# Autodesk Inventor assembly: head_v2
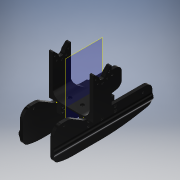
[picture p0: Inventor's stored thumbnail of the model, 180x180]
Saved by Autodesk Inventor 2018 (Build 220112000, 112)
## iProperties
Created: 2020-02-17
Part Number: head_v2
Document SubType Name: Assembly
Designer: bitbots
Author: bitbots
## Documents named in this file (4)
- C:\Users\bitbots\Desktop\bitbots_hardware\wolfgang\assembly\head\head_v2.iam
- C:\Users\bitbots\Desktop\bitbots_hardware\wolfgang\assembly\head\camera_lower_baseler_wolfgang_v2.1.ipt
- C:\Users\bitbots\Desktop\bitbots_hardware\wolfgang\assembly\head\camera_side_basler_wolfgang_v2.2.ipt
- C:\Users\bitbots\Desktop\bitbots_hardware\wolfgang\assembly\head\camera_side_basler_wolfgang_v2.2_MIR1.ipt
## Components (3 placed, 3 different names)
1. camera_lower_baseler_wolfgang_v2.1:1 — Mate:1, Mate:2, Mate:3, Flush:1, Mate:5, Mate:6, Mate:7, Mate:8, Mate:9, Mate:10
2. camera_side_basler_wolfgang_v2.2:1 — Mate:5, Mate:6, Mate:7
3. camera_side_basler_wolfgang_v2.2_MIR1:1 — Mate:8, Mate:9, Mate:10
## Relationships (11: Mate 10, Flush 1)
- Mate:1: camera_lower_baseler_wolfgang_v2.1:1
- Mate:2: camera_lower_baseler_wolfgang_v2.1:1
- Mate:3: camera_lower_baseler_wolfgang_v2.1:1
- Flush:1 (14.6 mm): camera_lower_baseler_wolfgang_v2.1:1
- Mate:4
- Mate:5: camera_lower_baseler_wolfgang_v2.1:1 ↔ camera_side_basler_wolfgang_v2.2:1
- Mate:6: camera_lower_baseler_wolfgang_v2.1:1 ↔ camera_side_basler_wolfgang_v2.2:1
- Mate:7: camera_lower_baseler_wolfgang_v2.1:1 ↔ camera_side_basler_wolfgang_v2.2:1
- Mate:8: camera_lower_baseler_wolfgang_v2.1:1 ↔ camera_side_basler_wolfgang_v2.2_MIR1:1
- Mate:9: camera_lower_baseler_wolfgang_v2.1:1 ↔ camera_side_basler_wolfgang_v2.2_MIR1:1
- Mate:10: camera_lower_baseler_wolfgang_v2.1:1 ↔ camera_side_basler_wolfgang_v2.2_MIR1:1
